# Autodesk Inventor assembly: 4xSplitter-Enclosure
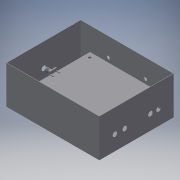
[picture p0: Inventor's stored thumbnail of the model, 180x180]
Saved by Autodesk Inventor 2018 (Build 220112000, 112)
## iProperties
Created: 2018-04-30
Part Number: 4xSplitter-Enclosure
Document SubType Name: Assembly
Designer: bbramman
Author: bbramman
## Documents named in this file (3)
- C:\Users\bbramman\OneDrive\Documents\Trapped Ion Research (Grad)\Electronics\pll-evalboard-synthesizer\Box CAD\4xSplitter-Enclosure.iam
- C:\Users\bbramman\OneDrive\Documents\Trapped Ion Research (Grad)\Electronics\pll-evalboard-synthesizer\Box CAD\563-AC-1404-4xSplitter.ipt
- C:\Users\bbramman\OneDrive\Documents\Trapped Ion Research (Grad)\Electronics\pll-evalboard-synthesizer\Box CAD\4xSplitter.iam
## Components (2 placed, 2 different names)
1. 563-AC-1404-4xSplitter:1 — Insert:1
2. 4xSplitter:1 [sub-assembly] — Insert:1
## Relationships (1: Insert 1)
- Insert:1 (19.05 mm): 563-AC-1404-4xSplitter:1 ↔ 4xSplitter:1
